# Autodesk Inventor assembly: LimeLight105
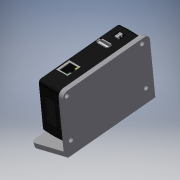
[picture p0: Inventor's stored thumbnail of the model, 180x180]
Saved by Autodesk Inventor 2019 (Build 230136000, 136)
## iProperties
Created: 2019-12-14
Part Number: LimeLight105
Document SubType Name: Assembly
Designer: james
Author: james
## Documents named in this file (3)
- F:\JimsRobot\FIRSTRobots\Design\Library\Jims\LimeLight105.iam
- F:\JimsRobot\FIRSTRobots\Design\Library\Jims\LimeLight120.ipt
- F:\JimsRobot\FIRSTRobots\Design\Library\LimeLight\LimelightCAD2STEPSimp.ipt
## Components (2 placed, 2 different names)
1. LimeLight120:1 — Mate:1, Mate:2, Mate:3
2. LimelightCAD2STEPSimp:1 — Mate:1, Mate:2, Mate:3
## Relationships (3: Mate 3)
- Mate:1: LimeLight120:1 ↔ LimelightCAD2STEPSimp:1
- Mate:2: LimeLight120:1 ↔ LimelightCAD2STEPSimp:1
- Mate:3: LimeLight120:1 ↔ LimelightCAD2STEPSimp:1
